# Autodesk Inventor assembly: UNOBatteryPack
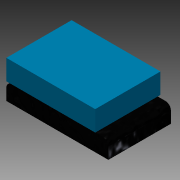
[picture p0: Inventor's stored thumbnail of the model, 180x180]
Saved by Autodesk Inventor 2014 SP1 (Build 180222100, 222)
## iProperties
Created: 2017-01-20
Part Number: UNOBatteryPack
Document SubType Name: Assembly
Designer: danielsikar
Author: danielsikar
## Documents named in this file (3)
- C:\Users\danielsikar\Documents\Inventor\IoT-Trike\Assemblies\UNOBatteryPack.iam
- C:\Users\danielsikar\Documents\Inventor\IoT-Trike\Parts\BatteryPack.ipt
- C:\Users\danielsikar\Documents\Inventor\IoT-Trike\Parts\UNO.ipt
## Components (2 placed, 2 different names)
1. BatteryPack:1 — Mate:1, Mate:2, Mate:3, Mate:4
2. UNO:1 — Mate:4, Mate:5, Mate:6
## Relationships (6: Mate 6)
- Mate:1: BatteryPack:1
- Mate:2: BatteryPack:1
- Mate:3: BatteryPack:1
- Mate:4: BatteryPack:1 ↔ UNO:1
- Mate:5: UNO:1
- Mate:6: UNO:1
